# Autodesk Inventor assembly: boardC
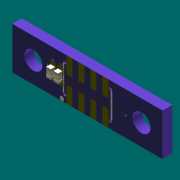
[picture p0: Inventor's stored thumbnail of the model, 180x180]
Saved by Autodesk Inventor 2016 SP1 (Build 200210100, 210)
## iProperties
Created: 2016-02-15
Part Number: boardC
Document SubType Name: Assembly
Designer: sawai
Author: sawai
## Documents named in this file (4)
- C:\Users\sawai\OneDrive\projects\mppcSensorInterface\cad\sensorBoardC\boardC.iam
- C:\Users\sawai\OneDrive\projects\mppcSensorInterface\cad\sensorBoardC\pcb.ipt
- C:\Users\sawai\OneDrive\projects\mppcSensorInterface\cad\electronics\capacitor-0603.ipt
- C:\Users\sawai\OneDrive\projects\mppcSensorInterface\cad\electronics\capacitor.ipt
## Components (3 placed, 2 different names)
1. pcb:1 — Mate:1
2. capacitor-0603:1 — Flush:1, Flush:2
3. capacitor-0603:2 — Flush:1, Flush:2, Mate:1
## Relationships (3: Flush 2, Mate 1)
- Flush:1: capacitor-0603:1 ↔ capacitor-0603:2
- Flush:2: capacitor-0603:1 ↔ capacitor-0603:2
- Mate:1: pcb:1 ↔ capacitor-0603:2
